# Autodesk Inventor assembly: Filament_Winder
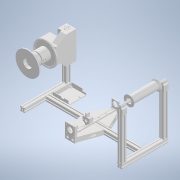
[picture p0: Inventor's stored thumbnail of the model, 180x180]
Saved by Autodesk Inventor 2021 (Build 250183000, 183)
## iProperties
Created: 2024-01-31
Part Number: Filament_Winder
Document SubType Name: Assembly
Designer: Lukas
Author: Lukas
## Documents named in this file (17)
- \\192.168.1.200\Storragepool\Datastorrage\Projects\Filament-Winder\Filament_Winder.iam
- \\192.168.1.200\Storragepool\Datastorrage\Projects\Filament-Winder\Profil.ipt
- \\192.168.1.200\Storragepool\Datastorrage\Projects\Filament-Winder\Gearmotor.ipt
- \\192.168.1.200\Storragepool\Datastorrage\Projects\Filament-Winder\Pulley.ipt
- \\192.168.1.200\Storragepool\Datastorrage\Projects\Filament-Winder\Motorhalterig.ipt
- \\192.168.1.200\Storragepool\Datastorrage\Projects\Filament-Winder\Gegestuck.ipt
- \\192.168.1.200\Storragepool\Datastorrage\Projects\Filament-Winder\Stengeli.ipt
- \\192.168.1.200\Storragepool\Datastorrage\Projects\Filament-Winder\Riiserolle.ipt
- \\192.168.1.200\Storragepool\Datastorrage\Projects\Filament-Winder\Verbinder.ipt
- \\192.168.1.200\Storragepool\Datastorrage\Projects\Filament-Winder\Stengelihalter.ipt
- \\192.168.1.200\Storragepool\Datastorrage\Projects\Filament-Winder\SliderMotorHalter.ipt
- \\192.168.1.200\Storragepool\Datastorrage\Projects\Filament-Winder\SliderLagerHalter.ipt
- \\192.168.1.200\Storragepool\Datastorrage\Projects\Filament-Winder\Rail.ipt
- \\192.168.1.200\Storragepool\Datastorrage\Projects\Filament-Winder\Slider.ipt
- \\192.168.1.200\Storragepool\Datastorrage\Projects\Filament-Winder\Guider.ipt
- \\192.168.1.200\Storragepool\Datastorrage\Projects\Filament-Winder\Endschalterhalter.ipt
- \\192.168.1.200\Storragepool\Datastorrage\Projects\Filament-Winder\Electronicsmount.ipt
## Components (23 placed, 16 different names)
1. Profil:1 — Mate:1, Flush:1, Flush:2, Mate:2, Flush:3, Flush:4, Flush:5, Flush:6, Mate:41, Flush:24, Flush:25
2. Profil:2 — Mate:1, Flush:1, Flush:2, Mate:6, Mate:7, Flush:12
3. Profil:3 — Mate:2, Flush:3, Flush:4, Mate:16, Flush:13, Flush:14, Mate:17, Mate:28, Flush:20, Mate:29
4. Profil:4 — Flush:5, Flush:6, Mate:13, Flush:7, Flush:8, Mate:14, Flush:9, Flush:10, Mate:20
5. Profil:5 — Mate:13, Flush:7, Flush:8, Mate:22, Mate:23, Flush:16
6. Profil:6 — Mate:14, Flush:9, Flush:10, Mate:21, Mate:24, Flush:15
7. Gearmotor:1 — Mate:4, Mate:5, Mate:8, Mate:15, Flush:11, Angle:1
8. Pulley:1 — Mate:4, Mate:5, Mate:10, Mate:11, Mate:12, Angle:1
9. Motorhalterig:1 — Mate:6, Mate:7, Mate:8, Mate:15, Flush:11, Flush:12
10. Gegestuck:1 — Mate:10, Mate:11, Mate:12
11. Stengeli:1 — Mate:25, Flush:17, Flush:18, Mate:26, Mate:27, Flush:19
12. Riiserolle:1 — Mate:26, Mate:27, Flush:19
13. Verbinder:1 — Mate:17, Mate:18, Mate:19
14. Profil:7 — Mate:16, Flush:13, Flush:14, Mate:18, Mate:19, Mate:20, Mate:30, Flush:21
15. Stengelihalter:1 — Mate:22, Mate:23, Flush:16, Mate:25, Flush:17, Flush:18
16. Stengelihalter:2 — Mate:21, Mate:24, Flush:15
17. SliderMotorHalter:1 — Mate:28, Flush:20, Mate:29, Flush:22, Mate:34, Flush:23, Mate:38, Mate:39, Mate:40
18. SliderLagerHalter:1 — Mate:30, Flush:21, Flush:22, Mate:31, Mate:32, Mate:33
19. Rail:1 — Mate:31, Mate:32, Mate:33
20. Slider:1 — Mate:34, Flush:23, Mate:35, Mate:36, Mate:37
21. Guider:1 — Mate:35, Mate:36, Mate:37
22. Endschalterhalter:1 — Mate:38, Mate:39, Mate:40
23. Electronicsmount:1 — Mate:41, Flush:24, Flush:25
## Relationships (65: Mate 39, Flush 25, Angle 1)
- Mate:1: Profil:1 ↔ Profil:2
- Flush:1: Profil:1 ↔ Profil:2
- Flush:2: Profil:1 ↔ Profil:2
- Mate:2: Profil:1 ↔ Profil:3
- Flush:3: Profil:1 ↔ Profil:3
- Flush:4: Profil:1 ↔ Profil:3
- Flush:5: Profil:1 ↔ Profil:4
- Flush:6: Profil:1 ↔ Profil:4
- Mate:4: Gearmotor:1 ↔ Pulley:1
- Mate:5 (1 mm): Gearmotor:1 ↔ Pulley:1
- Mate:6 (0.05 mm): Profil:2 ↔ Motorhalterig:1
- Mate:7 (0.05 mm): Profil:2 ↔ Motorhalterig:1
- Mate:8: Gearmotor:1 ↔ Motorhalterig:1
- Mate:10: Pulley:1 ↔ Gegestuck:1
- Mate:11: Pulley:1 ↔ Gegestuck:1
- Mate:12 (68 mm): Pulley:1 ↔ Gegestuck:1
- Mate:13: Profil:4 ↔ Profil:5
- Flush:7: Profil:4 ↔ Profil:5
- Flush:8: Profil:4 ↔ Profil:5
- Mate:14: Profil:4 ↔ Profil:6
- Flush:9: Profil:4 ↔ Profil:6
- Flush:10: Profil:4 ↔ Profil:6
- Mate:15 (0.1 mm): Gearmotor:1 ↔ Motorhalterig:1
- Flush:11 (2 mm): Gearmotor:1 ↔ Motorhalterig:1
- Flush:12: Profil:2 ↔ Motorhalterig:1
- Angle:1 (0 deg): Gearmotor:1 ↔ Pulley:1
- Mate:16: Profil:3 ↔ Profil:7
- Flush:13: Profil:3 ↔ Profil:7
- Flush:14: Profil:3 ↔ Profil:7
- Mate:17: Profil:3 ↔ Verbinder:1
- Mate:18: Verbinder:1 ↔ Profil:7
- Mate:19: Verbinder:1 ↔ Profil:7
- Mate:20: Profil:4 ↔ Profil:7
- Mate:21: Profil:6 ↔ Stengelihalter:2
- Mate:22: Profil:5 ↔ Stengelihalter:1
- Mate:23: Profil:5 ↔ Stengelihalter:1
- Mate:24: Profil:6 ↔ Stengelihalter:2
- Flush:15: Profil:6 ↔ Stengelihalter:2
- Flush:16: Profil:5 ↔ Stengelihalter:1
- Mate:25: Stengeli:1 ↔ Stengelihalter:1
- Flush:17: Stengeli:1 ↔ Stengelihalter:1
- Flush:18: Stengeli:1 ↔ Stengelihalter:1
- Mate:26: Stengeli:1 ↔ Riiserolle:1
- Mate:27: Stengeli:1 ↔ Riiserolle:1
- Flush:19: Stengeli:1 ↔ Riiserolle:1
- Mate:28: Profil:3 ↔ SliderMotorHalter:1
- Flush:20: Profil:3 ↔ SliderMotorHalter:1
- Mate:29: Profil:3 ↔ SliderMotorHalter:1
- Mate:30: Profil:7 ↔ SliderLagerHalter:1
- Flush:21: Profil:7 ↔ SliderLagerHalter:1
- Flush:22: SliderMotorHalter:1 ↔ SliderLagerHalter:1
- Mate:31: SliderLagerHalter:1 ↔ Rail:1
- Mate:32: SliderLagerHalter:1 ↔ Rail:1
- Mate:33: SliderLagerHalter:1 ↔ Rail:1
- Mate:34: SliderMotorHalter:1 ↔ Slider:1
- Flush:23: SliderMotorHalter:1 ↔ Slider:1
- Mate:35: Slider:1 ↔ Guider:1
- Mate:36: Slider:1 ↔ Guider:1
- Mate:37: Slider:1 ↔ Guider:1
- Mate:38: SliderMotorHalter:1 ↔ Endschalterhalter:1
- Mate:39: SliderMotorHalter:1 ↔ Endschalterhalter:1
- Mate:40: SliderMotorHalter:1 ↔ Endschalterhalter:1
- Mate:41: Profil:1 ↔ Electronicsmount:1
- Flush:24: Profil:1 ↔ Electronicsmount:1
- Flush:25: Profil:1 ↔ Electronicsmount:1
